# Autodesk Inventor assembly: demo
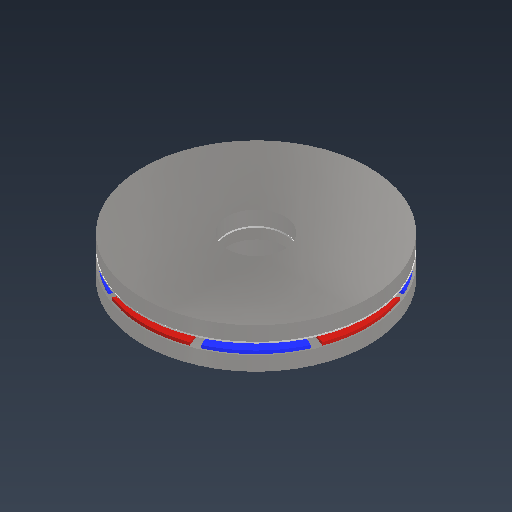
[picture p0: Inventor's stored thumbnail of the model, 512x512]
Saved by Autodesk Inventor 2025.3 (Build 293356000, 356)
## iProperties
Created: 2025-12-02
Part Number: demo
Document SubType Name: Assembly
Designer: 陳泓任
Author: 陳泓任
## Documents named in this file (4)
- C:\Users\Ou918\ECB_project\CAD\demo.iam
- C:\Users\Ou918\ECB_project\CAD\yield.ipt
- C:\Users\Ou918\ECB_project\CAD\magnet.ipt
- C:\Users\Ou918\ECB_project\CAD\conductor.ipt
## Components (11 placed, 3 different names)
1. yield:1 — concentricity_2, attach_2, 貼合:12, 貼合:13, 貼合:15, 貼合:16, 貼合:17, 貼合:18, 貼合:19, 貼合:20, 貼合:21, 貼合:22, 貼合:23, 貼合:24, 貼合:25, 貼合:26, 貼合:27, 貼合:28
2. magnet:1 — concentricity_2, attach_2, alignment, 角度:1
3. magnet:2 — 貼合:15, 貼合:22, 角度:1, 角度:2
4. magnet:3 — 貼合:20, 貼合:23, 角度:2, 角度:3
5. magnet:4 — 貼合:19, 貼合:26, 角度:3, 角度:4
6. magnet:5 — 貼合:18, 貼合:25, 角度:4, 角度:5
7. magnet:6 — 貼合:17, 貼合:24, 角度:5, 角度:6
8. magnet:7 — 貼合:16, 貼合:21, 角度:6, 角度:7
9. magnet:8 — 貼合:27, 貼合:28, 角度:7
10. conductor:1 — 貼合:12, 貼合:14
11. yield:2 — 貼合:13, 貼合:14
## Relationships (27: Mate 20, Angle 7)
- concentricity_2 [Mate]: yield:1 ↔ magnet:1
- attach_2 [Mate]: yield:1 ↔ magnet:1
- alignment [Mate]: magnet:1
- 貼合:12 [Mate]: yield:1 ↔ conductor:1
- 貼合:13 [Mate]: yield:1 ↔ yield:2
- 貼合:14 [Mate]: conductor:1 ↔ yield:2
- 貼合:15 [Mate]: yield:1 ↔ magnet:2
- 貼合:16 [Mate]: yield:1 ↔ magnet:7
- 貼合:17 [Mate]: yield:1 ↔ magnet:6
- 貼合:18 [Mate]: yield:1 ↔ magnet:5
- 貼合:19 [Mate]: yield:1 ↔ magnet:4
- 貼合:20 [Mate]: yield:1 ↔ magnet:3
- 貼合:21 [Mate]: yield:1 ↔ magnet:7
- 貼合:22 [Mate]: yield:1 ↔ magnet:2
- 貼合:23 [Mate]: yield:1 ↔ magnet:3
- 貼合:24 [Mate]: yield:1 ↔ magnet:6
- 貼合:25 [Mate]: yield:1 ↔ magnet:5
- 貼合:26 [Mate]: yield:1 ↔ magnet:4
- 貼合:27 [Mate]: yield:1 ↔ magnet:8
- 貼合:28 [Mate]: yield:1 ↔ magnet:8
- 角度:1 [Angle] (45 deg): magnet:1 ↔ magnet:2
- 角度:2 [Angle] (45 deg): magnet:2 ↔ magnet:3
- 角度:3 [Angle] (45 deg): magnet:3 ↔ magnet:4
- 角度:4 [Angle] (45 deg): magnet:4 ↔ magnet:5
- 角度:5 [Angle] (45 deg): magnet:5 ↔ magnet:6
- 角度:6 [Angle] (45 deg): magnet:6 ↔ magnet:7
- 角度:7 [Angle] (45 deg): magnet:7 ↔ magnet:8
## Named parameters: theta_p = 45 deg
